# Autodesk Inventor assembly: gantry_x
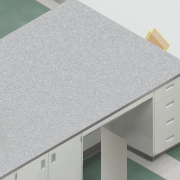
[picture p0: Inventor's stored thumbnail of the model, 180x180]
Saved by Autodesk Inventor 2016 SP2 (Build 200236200, 236)
## iProperties
Created: 2017-08-29
Part Number: gantry_x
Document SubType Name: Assembly
Designer: Admin
Author: Admin
## Documents named in this file (16)
- E:\DATA\Inventor\AtongJali_v2\gantry_x.iam
- E:\DATA\Inventor\AtongJali_v2\side_holder_R_1.ipt
- E:\DATA\Inventor\AtongJali_v2\side_load_R_1.ipt
- E:\DATA\Inventor\AtongJali_v2\holder_top_1.ipt
- E:\DATA\Inventor\AtongJali_v2\holder_base_1.ipt
- E:\DATA\Inventor\AtongJali_v2\holder_center_1.ipt
- E:\DATA\Inventor\AtongJali_v2\side_load_L_1.ipt
- E:\DATA\Inventor\AtongJali_v2\side_holder_L_1.ipt
- E:\DATA\Inventor\AtongJali_v2\pipa170.ipt
- E:\DATA\Inventor\AtongJali_v2\X-gan_holder.ipt
- E:\DATA\Inventor\AtongJali_v2\Linear_pipe.ipt
- E:\DATA\Inventor\AtongJali_v2\back_plate_gantry.ipt
- E:\DATA\Inventor\AtongJali_v2\front_plate_Z.ipt
- E:\DATA\Inventor\AtongJali_v2\Back_plate_Z.ipt
- E:\DATA\Inventor\AtongJali_v2\upper_block.ipt
- E:\DATA\Inventor\AtongJali_v2\Lower_wheel.iam
## Components (20 placed, 15 different names)
1. side_holder_R_1:1 — Flush:8
2. side_load_R_1:1
3. holder_top_1:1
4. holder_base_1:1
5. holder_center_1:1
6. side_load_L_1:1
7. side_holder_L_1:1 — Rotational:1, Rotational:2
8. pipa170:1 — Rotational:1, Rotational:3, Cylindrical:1, Cylindrical:4, Cylindrical:3
9. pipa170:2 — Rotational:2, Cylindrical:2, Cylindrical:5, Cylindrical:6
10. X-gan_holder:1 — Rotational:3, Mate:2
11. X-gan_holder:2 — Cylindrical:1, Cylindrical:2, Mate:2, Rigid:1
12. Linear_pipe:1 — Cylindrical:4, Flush:1, Mate:1, Flush:3, Rotational:4
13. Linear_pipe:2 — Cylindrical:3, Flush:1, Mate:1, Flush:4, Flush:5, Rotational:5, Rotational:6
14. Linear_pipe:3 — Cylindrical:5, Flush:2, Flush:3
15. Linear_pipe:4 — Cylindrical:6, Flush:2, Flush:4, Flush:5
16. back_plate_gantry:1 — Flush:8
17. front_plate_Z:1 — Rotational:4, Rotational:5, Flush:9
18. Back_plate_Z:1 — Rotational:6, Flush:9
19. upper_block:1 — Rigid:1, Mate:3, Flush:10
20. Lower_wheel:1 [sub-assembly] — Mate:3, Flush:10
## Relationships (24: Flush 8, RevoluteJoint 6, CylindricalJoint 6, Mate 3, WeldJoint 1)
- Rotational:1 [RevoluteJoint]: side_holder_L_1:1 ↔ pipa170:1
- Rotational:2 [RevoluteJoint]: side_holder_L_1:1 ↔ pipa170:2
- Rotational:3 [RevoluteJoint]: pipa170:1 ↔ X-gan_holder:1
- Cylindrical:1: pipa170:1 ↔ X-gan_holder:2
- Cylindrical:2: pipa170:2 ↔ X-gan_holder:2
- Cylindrical:4: pipa170:1 ↔ Linear_pipe:1
- Cylindrical:3: pipa170:1 ↔ Linear_pipe:2
- Cylindrical:5: pipa170:2 ↔ Linear_pipe:3
- Cylindrical:6: pipa170:2 ↔ Linear_pipe:4
- Flush:1: Linear_pipe:1 ↔ Linear_pipe:2
- Flush:2: Linear_pipe:3 ↔ Linear_pipe:4
- Mate:1 (10 mm): Linear_pipe:1 ↔ Linear_pipe:2
- Flush:3: Linear_pipe:1 ↔ Linear_pipe:3
- Flush:4: Linear_pipe:2 ↔ Linear_pipe:4
- Flush:5: Linear_pipe:2 ↔ Linear_pipe:4
- Flush:8: side_holder_R_1:1 ↔ back_plate_gantry:1
- Rotational:4 [RevoluteJoint]: Linear_pipe:1 ↔ front_plate_Z:1
- Rotational:5 [RevoluteJoint]: Linear_pipe:2 ↔ front_plate_Z:1
- Rotational:6 [RevoluteJoint]: Linear_pipe:2 ↔ Back_plate_Z:1
- Flush:9: front_plate_Z:1 ↔ Back_plate_Z:1
- Mate:2 (50 mm): X-gan_holder:1 ↔ X-gan_holder:2
- Rigid:1 [WeldJoint]: X-gan_holder:2 ↔ upper_block:1
- Mate:3 (15 mm): upper_block:1 ↔ Lower_wheel:1
- Flush:10: upper_block:1 ↔ Lower_wheel:1
